# Autodesk Inventor assembly: Print Assembly
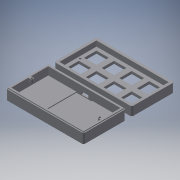
[picture p0: Inventor's stored thumbnail of the model, 180x180]
Saved by Autodesk Inventor 2018 (Build 220112000, 112)
## iProperties
Created: 2018-05-10
Part Number: Print Assembly
Document SubType Name: Assembly
Designer: mtsti
Author: mtsti
## Documents named in this file (3)
- C:\Users\mtsti\Desktop\Macro Deck\Print Assembly.iam
- C:\Users\mtsti\Desktop\Macro Deck\Base.ipt
- C:\Users\mtsti\Desktop\Macro Deck\Key Plate.ipt
## Components (2 placed, 2 different names)
1. Base:1 — Flush:1, Flush:2
2. Key Plate:1 — Flush:1, Flush:2
## Relationships (2: Flush 2)
- Flush:1: Base:1 ↔ Key Plate:1
- Flush:2: Base:1 ↔ Key Plate:1
